# Autodesk Inventor assembly: mascon-new
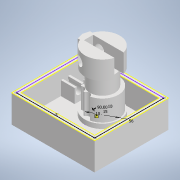
[picture p0: Inventor's stored thumbnail of the model, 180x180]
Saved by Autodesk Inventor 2021 (Build 250183000, 183)
## iProperties
Created: 2021-04-28
Part Number: mascon-new
Document SubType Name: Assembly
Designer: ben
Author: ben
## Documents named in this file (4)
- C:\Users\teh18\OneDrive\BVE Controller\r68-bve-mascon\mascon-new.iam
- C:\Users\teh18\OneDrive\BVE Controller\r68-bve-mascon\mascon.ipt
- C:\Users\teh18\OneDrive\BVE Controller\r68-bve-mascon\handle_base.ipt
- C:\Users\teh18\OneDrive\BVE Controller\r68-bve-mascon\handle_base2.ipt
## Components (3 placed, 3 different names)
1. mascon:1 — Rotational:1
2. handle_base:1 — Rotational:1, Flush:1
3. handle_base2:1 — Flush:1
## Relationships (2: RevoluteJoint 1, Flush 1)
- Rotational:1 [RevoluteJoint]: mascon:1 ↔ handle_base:1
- Flush:1: handle_base:1 ↔ handle_base2:1
